# Autodesk Inventor assembly: HbSensorU01
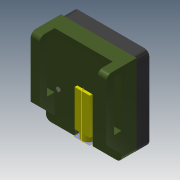
[picture p0: Inventor's stored thumbnail of the model, 180x180]
Saved by Autodesk Inventor 2015 SP1 (Build 190203100, 203)
## iProperties
Created: 2015-05-21
Part Number: HbSensorU01
Document SubType Name: Assembly
Designer: Yamaura
Title: export2
Description: Alibre Inc.
Creation Date: 2015-05-21
Sending System: Alibre
Preprocessor: ST-DEVELOPER v14
Author: Yamaura
## Documents named in this file (7)
- C:\Users\Yamaura\Google ドライブ\exiii\3D\150405HackBerry\00_Latest\Imported Components\HbSensorU01\HbSensorU01.iam
- C:\Users\Yamaura\Google ドライブ\exiii\3D\150405HackBerry\00_Latest\HbSensorHolder01.ipt
- C:\Users\Yamaura\Google ドライブ\exiii\3D\150405HackBerry\00_Latest\HbSensorBoard01.ipt
- C:\Users\Yamaura\Google ドライブ\exiii\3D\150405HackBerry\00_Latest\Imported Components\TPR-105\TPR-105.ipt
- C:\Users\Yamaura\Google ドライブ\exiii\3D\150405HackBerry\00_Latest\MJ-4535-3.ipt
- C:\Users\Yamaura\Google ドライブ\exiii\3D\150405HackBerry\00_Latest\ScrewM2L6.ipt
- C:\Users\Yamaura\Google ドライブ\exiii\3D\150405HackBerry\00_Latest\HbSensorCushion01.ipt
## Components (7 placed, 6 different names)
1. HbSensorHolder01:1 — フラッシュ:1, メイト:7, メイト:8
2. HbSensorBoard01:1 — メイト:1, メイト:2, メイト:3, メイト:4, メイト:5, メイト:6, メイト:11
3. TPR-105:1 — メイト:1, メイト:2, 角度:1
4. MJ-4535-3:1 — メイト:3, フラッシュ:2, メイト:4
5. ScrewM2L6:1 — メイト:5, メイト:7
6. ScrewM2L6:2 — メイト:6, メイト:8
7. HbSensorCushion01:1 — メイト:9, メイト:10, メイト:11
## Relationships (14: Mate 11, Flush 2, Angle 1)
- フラッシュ:1 [Flush]: HbSensorHolder01:1
- メイト:1 [Mate]: HbSensorBoard01:1 ↔ TPR-105:1
- メイト:2 [Mate]: HbSensorBoard01:1 ↔ TPR-105:1
- 角度:1 [Angle] (90 deg): TPR-105:1
- メイト:3 [Mate]: HbSensorBoard01:1 ↔ MJ-4535-3:1
- フラッシュ:2 [Flush]: MJ-4535-3:1
- メイト:4 [Mate]: HbSensorBoard01:1 ↔ MJ-4535-3:1
- メイト:5 [Mate]: HbSensorBoard01:1 ↔ ScrewM2L6:1
- メイト:6 [Mate]: HbSensorBoard01:1 ↔ ScrewM2L6:2
- メイト:7 [Mate]: HbSensorHolder01:1 ↔ ScrewM2L6:1
- メイト:8 [Mate]: HbSensorHolder01:1 ↔ ScrewM2L6:2
- メイト:9 [Mate]: HbSensorCushion01:1
- メイト:10 [Mate]: HbSensorCushion01:1
- メイト:11 [Mate]: HbSensorBoard01:1 ↔ HbSensorCushion01:1
